# Autodesk Inventor assembly: Assembly_V6
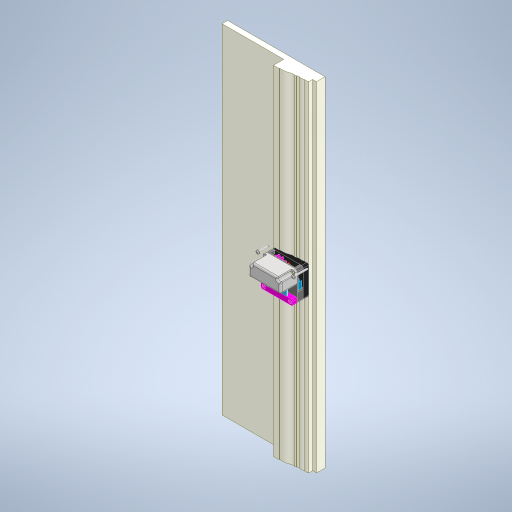
[picture p0: Inventor's stored thumbnail of the model, 512x512]
Saved by Autodesk Inventor 2023 (Build 270158000, 158)
## iProperties
Created: 2023-03-15
Part Number: Assembly_V6
Document SubType Name: Assembly
Designer: shrey
Author: shrey
## Documents named in this file (15)
- D:\Inventor Projects\Door Lock\V6\Assembly_V6.iam
- D:\Inventor Projects\Door Lock\V4\moulding.ipt
- D:\Inventor Projects\Door Lock\motor.ipt
- D:\Inventor Projects\Door Lock\V6\Assembly_V6\Design Accelerator\Spur Gears1.iam
- D:\Inventor Projects\Door Lock\V6\pinion_V6.ipt
- D:\Inventor Projects\Door Lock\V6\rack_V6.ipt
- D:\Inventor Projects\Door Lock\V6\mouldingPlate_V6.ipt
- D:\Inventor Projects\Door Lock\V6\house_V6.ipt
- D:\Inventor Projects\Door Lock\V4\screw.ipt
- D:\Inventor Projects\Door Lock\V7\longerScrew.ipt
- D:\Inventor Projects\Door Lock\V7\connectorHolder.ipt
- D:\Inventor Projects\Door Lock\JST - XH - Thru (V) - 4Pin - 2.54mm.ipt
- D:\Inventor Projects\Door Lock\V6\ESP-12F.ipt
- D:\Inventor Projects\Door Lock\V6\pinion_nohole_V6.ipt
- D:\Inventor Projects\Door Lock\V6\motorCover_V6.ipt
## Components (16 placed, 14 different names)
1. moulding:1 — Flush:1, Flush:21, Flush:35, Flush:45
2. motor:1 — Mate:6, Mate:29, Mate:30, Flush:34, Mate:36, Mate:41
3. motor:2 — Mate:4, Flush:32, Flush:34, Flush:39, Mate:39, Mate:41
4. Spur Gears:1 [sub-assembly]
5. pinion_V6:1 — Mate:4, Mate:14, Mate:35
6. pinion_V6:2 — Mate:6, Flush:36, Mate:36, Mate:38
7. rack_V6:1 — Mate:42, Mate:43
8. mouldingPlate_V6:1 — Mate:12, Mate:13, Flush:6, Mate:14, Flush:10, Mate:18, Flush:13, Flush:14, Flush:42, Flush:43, Flush:45
9. house_V6:1 — Mate:16, Mate:17, Flush:9, Flush:10, Flush:11, Flush:40, Mate:37, Flush:39, Mate:40, Mate:42, Mate:43, Mate:45
10. screw:1 — Mate:18, Flush:11, Flush:44
11. longerScrew:1 — Flush:13, Flush:14
12. connectorHolder:1 — Mate:23, Mate:24, Mate:37, Flush:41
13. JST - XH - Thru (V) - 4Pin - 2.54mm:1 — Flush:40, Mate:40, Flush:41
14. ESP-12F:1
15. pinion_nohole_V6:1 — Mate:38, Mate:39
16. motorCover_V6:1 — Mate:44, Flush:42, Flush:43, Mate:45, Flush:44
## Relationships (42: Mate 23, Flush 19)
- Flush:1: moulding:1
- Mate:4: motor:2 ↔ pinion_V6:1
- Mate:6: motor:1 ↔ pinion_V6:2
- Mate:12: mouldingPlate_V6:1
- Mate:13: mouldingPlate_V6:1
- Flush:6: mouldingPlate_V6:1
- Mate:14: pinion_V6:1 ↔ mouldingPlate_V6:1
- Mate:16: house_V6:1
- Mate:17: house_V6:1
- Flush:9: house_V6:1
- Flush:10: mouldingPlate_V6:1 ↔ house_V6:1
- Mate:18 (-3 mm): mouldingPlate_V6:1 ↔ screw:1
- Flush:11: house_V6:1 ↔ screw:1
- Flush:13: mouldingPlate_V6:1 ↔ longerScrew:1
- Flush:14: mouldingPlate_V6:1 ↔ longerScrew:1
- Mate:23: connectorHolder:1
- Mate:24: connectorHolder:1
- Flush:40 (28.594 mm): house_V6:1 ↔ JST - XH - Thru (V) - 4Pin - 2.54mm:1
- Flush:21 (-28.594 mm): moulding:1
- Mate:29 (9 mm): motor:1
- Mate:30 (10 mm): motor:1
- Flush:32 (9 mm): motor:2
- Flush:34: motor:1 ↔ motor:2
- Flush:35 (-0.885 mm): moulding:1
- Flush:36 (-37.594 mm): pinion_V6:2
- Mate:35 (19.594 mm): pinion_V6:1
- Mate:36: motor:1 ↔ pinion_V6:2
- Mate:37: house_V6:1 ↔ connectorHolder:1
- Flush:39: motor:2 ↔ house_V6:1
- Mate:38 (1 mm): pinion_V6:2 ↔ pinion_nohole_V6:1
- Mate:39: motor:2 ↔ pinion_nohole_V6:1
- Mate:40: house_V6:1 ↔ JST - XH - Thru (V) - 4Pin - 2.54mm:1
- Flush:41: connectorHolder:1 ↔ JST - XH - Thru (V) - 4Pin - 2.54mm:1
- Mate:41: motor:1 ↔ motor:2
- Mate:42: rack_V6:1 ↔ house_V6:1
- Mate:43: rack_V6:1 ↔ house_V6:1
- Mate:44: motorCover_V6:1
- Flush:42: mouldingPlate_V6:1 ↔ motorCover_V6:1
- Flush:43: mouldingPlate_V6:1 ↔ motorCover_V6:1
- Mate:45: house_V6:1 ↔ motorCover_V6:1
- Flush:44: screw:1 ↔ motorCover_V6:1
- Flush:45: moulding:1 ↔ mouldingPlate_V6:1
